# Autodesk Inventor assembly: Arm
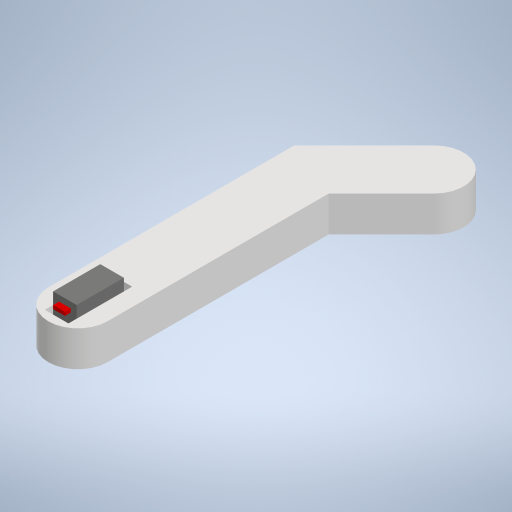
[picture p0: Inventor's stored thumbnail of the model, 512x512]
Saved by Autodesk Inventor 2023 (Build 270158000, 158)
## iProperties
Created: 2024-06-28
Part Number: Arm
Document SubType Name: Assembly
Designer: Swoby
Author: Swoby
## Documents named in this file (4)
- C:\Users\Swoby\OneDrive\Plocha\DUM-E\V0.2\Arm.iam
- C:\Users\Swoby\OneDrive\Plocha\DUM-E\V0.2\Servo_bigg_maketa.ipt
- C:\Users\Swoby\OneDrive\Plocha\DUM-E\V0.2\Servo_bigg_top.ipt
- C:\Users\Swoby\OneDrive\Plocha\DUM-E\V0.2\Arm 1 .ipt
## Components (3 placed, 3 different names)
1. Servo_bigg_maketa:1 — Mate:1, Mate:2, Mate:3, Mate:4
2. Servo_bigg_top:1 — Mate:4
3. Arm 1 :1 — Mate:1, Mate:2, Mate:3
## Relationships (4: Mate 4)
- Mate:1: Servo_bigg_maketa:1 ↔ Arm 1 :1
- Mate:2: Servo_bigg_maketa:1 ↔ Arm 1 :1
- Mate:3: Servo_bigg_maketa:1 ↔ Arm 1 :1
- Mate:4: Servo_bigg_maketa:1 ↔ Servo_bigg_top:1
